# Autodesk Inventor assembly: case-motor
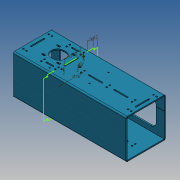
[picture p0: Inventor's stored thumbnail of the model, 180x180]
Saved by Autodesk Inventor 2017 (Build 210142000, 142)
## iProperties
Part Number: case-motor
Material: Genérico
Document SubType Name: Assembly
Designer: Leo
Author: Leo
## Documents named in this file (4)
- C:\Users\Leo\Documents\GitHub\actor-re-actor\3d\case-motor.iam
- C:\Users\Leo\Dropbox\E\Caja Motriz\Case\Protector.ipt
- C:\Users\Leo\Dropbox\E\Caja Motriz\Case\CaseB.ipt
- C:\Users\Leo\Dropbox\E\Caja Motriz\Case\Refuerzo U.ipt
## Components (3 placed, 3 different names)
1. CaseB:1 — Coincidencia:1, Nivelación:5
2. Protector:1 — Nivelación:1, Nivelación:2, Nivelación:3
3. Refuerzo U:1 — Nivelación:4, Coincidencia:1, Nivelación:5
## Relationships (6: Flush 5, Mate 1)
- Nivelación:1 [Flush] (40 mm): Protector:1
- Nivelación:2 [Flush]: Protector:1
- Nivelación:3 [Flush]: Protector:1
- Nivelación:4 [Flush]: Refuerzo U:1
- Coincidencia:1 [Mate]: CaseB:1 ↔ Refuerzo U:1
- Nivelación:5 [Flush]: CaseB:1 ↔ Refuerzo U:1
